# Autodesk Inventor assembly: innerHousingAssembly
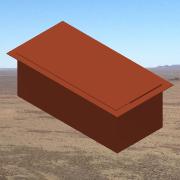
[picture p0: Inventor's stored thumbnail of the model, 180x180]
Saved by Autodesk Inventor 2014 SP1 (Build 180222100, 222)
## iProperties
Created: 2014-05-23
Part Number: innerHousingAssembly
Document SubType Name: Assembly
Designer: Dave
Author: Dave
## Documents named in this file (3)
- C:\Users\Dave\Desktop\hera-cad\Node\innerHousingAssembly.iam
- C:\Users\Dave\Desktop\hera-cad\Node\innerHousingBody.ipt
- C:\Users\Dave\Desktop\hera-cad\Node\innerHousingPlate.ipt
## Components (2 placed, 2 different names)
1. innerHousingBody:1 — Mate:1
2. innerHousingPlate:1 — Mate:1
## Relationships (1: Mate 1)
- Mate:1: innerHousingBody:1 ↔ innerHousingPlate:1
